# Autodesk Inventor assembly: SensoredMotor
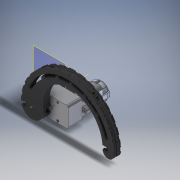
[picture p0: Inventor's stored thumbnail of the model, 180x180]
Saved by Autodesk Inventor 2016 (Build 200138000, 138)
## iProperties
Created: 2016-11-06
Part Number: SensoredMotor
Document SubType Name: Assembly
Designer: brent
Author: brent
## Documents named in this file (7)
- C:\Users\brent\OneDrive\classes\desinv22\final\leggedbot_mechanical\SensoredMotor.iam
- C:\Users\brent\OneDrive\classes\desinv22\final\leggedbot_mechanical\offtheshelf\AS5048B_Breakout.ipt
- C:\Users\brent\OneDrive\classes\desinv22\final\leggedbot_mechanical\offtheshelf\Pololu_120to1Offset.ipt
- C:\Users\brent\OneDrive\classes\desinv22\final\leggedbot_mechanical\offtheshelf\DiametricMagnet_625.ipt
- C:\Users\brent\OneDrive\classes\desinv22\final\leggedbot_mechanical\MagnetHolder.ipt
- C:\Users\brent\OneDrive\classes\desinv22\final\leggedbot_mechanical\EncoderMount.ipt
- C:\Users\brent\OneDrive\classes\desinv22\final\leggedbot_mechanical\Leg.ipt
## Components (6 placed, 6 different names)
1. AS5048B_Breakout:1 — Mate:2, Angle:1, Mate:3
2. Pololu_120to1Offset:1 — Flush:5, Flush:1, Mate:2, Angle:1, Mate:3, Mate:4, Mate:5, Flush:2, Flush:3, Flush:4, Mate:6, Mate:7
3. DiametricMagnet_625:1 — Mate:4, Mate:5
4. MagnetHolder:1 — Flush:2
5. EncoderMount:1 — Flush:3, Flush:4
6. Leg:1 — Mate:6, Mate:7
## Relationships (12: Mate 6, Flush 5, Angle 1)
- Flush:5: Pololu_120to1Offset:1
- Flush:1: Pololu_120to1Offset:1
- Mate:2: AS5048B_Breakout:1 ↔ Pololu_120to1Offset:1
- Angle:1 (0 deg): AS5048B_Breakout:1 ↔ Pololu_120to1Offset:1
- Mate:3 (3.5 mm): AS5048B_Breakout:1 ↔ Pololu_120to1Offset:1
- Mate:4: Pololu_120to1Offset:1 ↔ DiametricMagnet_625:1
- Mate:5: Pololu_120to1Offset:1 ↔ DiametricMagnet_625:1
- Flush:2: Pololu_120to1Offset:1 ↔ MagnetHolder:1
- Flush:3: Pololu_120to1Offset:1 ↔ EncoderMount:1
- Flush:4: Pololu_120to1Offset:1 ↔ EncoderMount:1
- Mate:6: Pololu_120to1Offset:1 ↔ Leg:1
- Mate:7 (0.5 mm): Pololu_120to1Offset:1 ↔ Leg:1
